# Autodesk Inventor assembly: CollectionProto
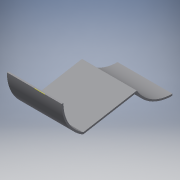
[picture p0: Inventor's stored thumbnail of the model, 180x180]
Saved by Autodesk Inventor 2019 (Build 230136000, 136)
## iProperties
Created: 2018-10-04
Part Number: CollectionProto
Document SubType Name: Assembly
Designer: User
Author: User
## Documents named in this file (3)
- C:\Robotics\CAD\2018-19_CAD\Collection\CollectionProto.iam
- C:\Robotics\CAD\2018-19_CAD\Collection\CollectorFloor.ipt
- C:\Robotics\CAD\2018-19_CAD\Collection\CollectorSweeperBacking.ipt
## Components (3 placed, 2 different names)
1. CollectorFloor:1 — Mate:2, Mate:3, Angle:1, Angle:2, Flush:1, Flush:2, Angle:3
2. CollectorSweeperBacking:1 — Mate:3, Angle:2, Flush:2
3. CollectorSweeperBacking:2 — Mate:2, Angle:1, Flush:1, Mate:1
## Relationships (8: Mate 3, Angle 3, Flush 2)
- Mate:1: CollectorSweeperBacking:2
- Mate:2: CollectorFloor:1 ↔ CollectorSweeperBacking:2
- Mate:3: CollectorFloor:1 ↔ CollectorSweeperBacking:1
- Angle:1 (-10 deg): CollectorFloor:1 ↔ CollectorSweeperBacking:2
- Angle:2 (100 deg): CollectorFloor:1 ↔ CollectorSweeperBacking:1
- Flush:1: CollectorFloor:1 ↔ CollectorSweeperBacking:2
- Flush:2: CollectorFloor:1 ↔ CollectorSweeperBacking:1
- Angle:3 (-10 deg): CollectorFloor:1
